# Autodesk Inventor assembly: FullSystemV01
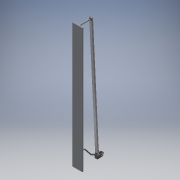
[picture p0: Inventor's stored thumbnail of the model, 180x180]
Saved by Autodesk Inventor 2016 (Build 200138000, 138)
## iProperties
Created: 2016-11-14
Part Number: FullSystemV01
Document SubType Name: Assembly
Designer: Matt Cocca
Author: Matt Cocca
## Documents named in this file (7)
- C:\Users\mattc\OneDrive\Documents\Inventor\EmbeddedBalance\Models\V01\FullSystemV01.iam
- C:\Users\mattc\OneDrive\Documents\Inventor\EmbeddedBalance\Models\V01\Base.ipt
- C:\Users\mattc\OneDrive\Documents\Inventor\EmbeddedBalance\Models\V01\ArmSpan.ipt
- C:\Users\mattc\OneDrive\Documents\Inventor\EmbeddedBalance\Models\V01\ServoLinkage.ipt
- C:\Users\mattc\OneDrive\Documents\Inventor\EmbeddedBalance\Models\V01\General_Parts\Track.ipt
- C:\Users\mattc\OneDrive\Documents\Inventor\EmbeddedBalance\Models\V01\TrackPivotConnector.ipt
- C:\Users\mattc\OneDrive\Documents\Inventor\EmbeddedBalance\Models\V01\General_Parts\EndStopGeneric.ipt
## Components (7 placed, 6 different names)
1. Base:1 — Insert:1, Insert:4
2. ServoLinkage:1 — Insert:1, Insert:2
3. ArmSpan:1 — Insert:2, Insert:3
4. Track:1 — Mate:1, Flush:1, Mate:2, Mate:3, Mate:4, Mate:6, Flush:2, Flush:3
5. TrackPivotConnector:1 — Mate:1, Flush:1, Mate:5, Insert:3
6. EndStopGeneric:1 — Mate:2, Mate:3, Mate:4, Mate:5
7. TrackPivotConnector:2 — Mate:6, Flush:2, Flush:3, Insert:4
## Relationships (13: Mate 6, Insert 4, Flush 3)
- Insert:1: Base:1 ↔ ServoLinkage:1
- Insert:2: ServoLinkage:1 ↔ ArmSpan:1
- Mate:1: Track:1 ↔ TrackPivotConnector:1
- Flush:1: Track:1 ↔ TrackPivotConnector:1
- Mate:2: Track:1 ↔ EndStopGeneric:1
- Mate:3: Track:1 ↔ EndStopGeneric:1
- Mate:4 (0.255 mm): Track:1 ↔ EndStopGeneric:1
- Mate:5: TrackPivotConnector:1 ↔ EndStopGeneric:1
- Insert:3: ArmSpan:1 ↔ TrackPivotConnector:1
- Mate:6: Track:1 ↔ TrackPivotConnector:2
- Flush:2: Track:1 ↔ TrackPivotConnector:2
- Flush:3: Track:1 ↔ TrackPivotConnector:2
- Insert:4: Base:1 ↔ TrackPivotConnector:2
